# Autodesk Inventor assembly: SE. fuente
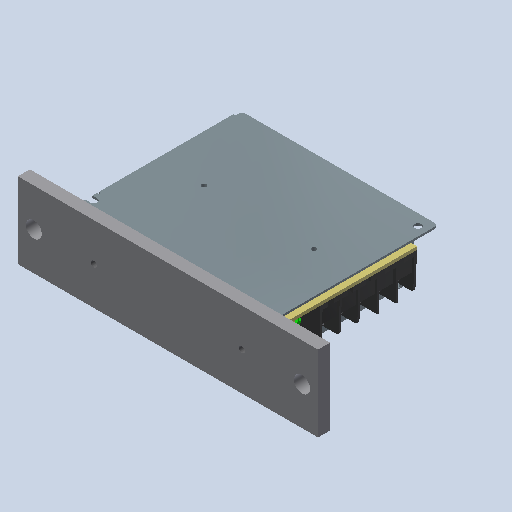
[picture p0: Inventor's stored thumbnail of the model, 512x512]
Saved by Autodesk Inventor 2024.2 (Build 282272000, 272)
## iProperties
Created: 2025-06-19
Part Number: SE. fuente
Material: Genérico
Document SubType Name: Assembly
Designer: jd.castellanosq
Author: jd.castellanosq
## Documents named in this file (3)
- I:\MICROMECANICA\ALTAS ENERGIAS\Deteccion de Muones\Detectores centelladores\Partes Detector Centellador\SE Chasis DC\Partes Chasis DC\SE. fuente.iam
- I:\MICROMECANICA\ALTAS ENERGIAS\Deteccion de Muones\Detectores centelladores\Partes Detector Centellador\SE Chasis DC\Partes Chasis DC\Soporte fuente.ipt
- I:\MICROMECANICA\ALTAS ENERGIAS\Deteccion de Muones\Detectores centelladores\Partes Detector Centellador\SE Tarjetas IC DC\Fuentes DC\Fuente DC.ipt
## Components (2 placed, 2 different names)
1. Soporte fuente:1 — Mate:1, Flush:1, Mate:2, Mate:3, Mate:4, Mate:5
2. Fuente DC:1 — Mate:3, Mate:4, Mate:5
## Relationships (6: Mate 5, Flush 1)
- Mate:1: Soporte fuente:1
- Flush:1: Soporte fuente:1
- Mate:2: Soporte fuente:1
- Mate:3: Soporte fuente:1 ↔ Fuente DC:1
- Mate:4: Soporte fuente:1 ↔ Fuente DC:1
- Mate:5: Soporte fuente:1 ↔ Fuente DC:1
